# Autodesk Inventor assembly: sled plexi
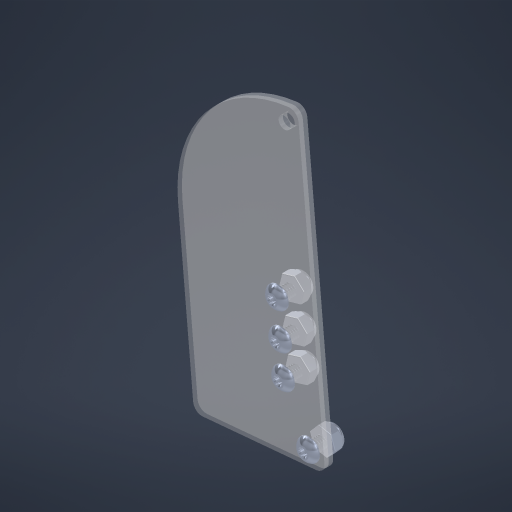
[picture p0: Inventor's stored thumbnail of the model, 512x512]
Saved by Autodesk Inventor 2023 (Build 270158000, 158)
## iProperties
Created: 2023-08-07
Part Number: sled plexi
Document SubType Name: Assembly
Designer: srbel
Author: srbel
## Documents named in this file (5)
- C:\CAD\OverUnderCAD\Drive\sled plexi.iam
- C:\CAD Robotics Season 23-24\sleds.ipt
- C:\CAD\OverUnderCAD\VEX-CAD-Inventor-1.4.0\Structure\Hardware\Screw Steel - Star.ipt
- C:\CAD\OverUnderCAD\VEX-CAD-Inventor-1.4.0\Structure\Hardware\Screw Steel - Star\SScrew Star Threaded .290.ipt
- C:\CAD\OverUnderCAD\VEX-CAD-Inventor-1.4.0\Structure\Hardware\Nut Thin Nylock.ipt
## Components (10 placed, 3 different names)
1. sleds:1 — Insert:1, Insert:2, Insert:6, Insert:8, Insert:9, Insert:12, Insert:17
2. sleds:2 — Insert:1, Insert:2, Insert:13, Insert:14, Insert:15, Insert:16, Insert:17
3. SScrew Star Threaded .290:10 — Insert:6
4. SScrew Star Threaded .290:11 — Insert:12
5. SScrew Star Threaded .290:13 — Insert:8
6. SScrew Star Threaded .290:14 — Insert:9
7. Nut Thin Nylock:1 — Insert:13
8. Nut Thin Nylock:2 — Insert:14
9. Nut Thin Nylock:4 — Insert:16
10. Nut Thin Nylock:7 — Insert:15
## Relationships (11: Insert 11)
- Insert:1: sleds:1 ↔ sleds:2
- Insert:2: sleds:1 ↔ sleds:2
- Insert:6: sleds:1 ↔ SScrew Star Threaded .290:10
- Insert:8: sleds:1 ↔ SScrew Star Threaded .290:13
- Insert:9: sleds:1 ↔ SScrew Star Threaded .290:14
- Insert:12: sleds:1 ↔ SScrew Star Threaded .290:11
- Insert:13 (1.5875 mm): sleds:2 ↔ Nut Thin Nylock:1
- Insert:14 (1.5875 mm): sleds:2 ↔ Nut Thin Nylock:2
- Insert:15 (1.5875 mm): sleds:2 ↔ Nut Thin Nylock:7
- Insert:16 (1.5875 mm): sleds:2 ↔ Nut Thin Nylock:4
- Insert:17: sleds:1 ↔ sleds:2
